# Autodesk Inventor assembly: Winch Assembly
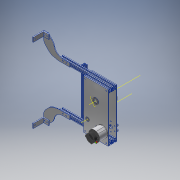
[picture p0: Inventor's stored thumbnail of the model, 180x180]
Saved by Autodesk Inventor 2019.4 (Build 234330000, 330)
## iProperties
Created: 2020-01-24
Part Number: Winch Assembly
Document SubType Name: Assembly
Designer: Mark
Mass: 3605.21 g
Surface Area: 5054.36 cm^2
Volume: 1017.6 cm^3
Density: 3.54284 g/cm^3
Author: Mark
## Documents named in this file (25)
- C:\Users\admin\Desktop\FRC 2020 Engineering\GitHub\7738-2020\Ratchet Winch\Winch Assembly.iam
- C:\Users\admin\Desktop\FRC 2020 Engineering\GitHub\7738-2020\Ratchet Winch\An Extrusion.ipt
- C:\Users\admin\Desktop\FRC 2020 Engineering\GitHub\7738-2020\Elevator MK2\Bottom Pneumatic Extrusion.ipt
- C:\Users\admin\Desktop\FRC 2020 Engineering\GitHub\7738-2020\Ratchet Winch\Support Plate.ipt
- C:\Users\admin\Desktop\FRC 2020 Engineering\GitHub\7738-2020\Ratchet Winch\Small connector.ipt
- C:\Users\admin\Desktop\FRC 2020 Engineering\GitHub\7738-2020\Ratchet Winch\V2 Plate 1.ipt
- C:\Users\admin\Desktop\FRC 2020 Engineering\GitHub\7738-2020\Ratchet Winch\Falcon_500_Powered_by_Talon_FX_217-6515.ipt
- C:\Users\admin\Desktop\FRC 2020 Engineering\GitHub\7738-2020\Robot V2\Turret\F6800.ipt
- C:\Users\admin\Desktop\FRC 2020 Engineering\GitHub\7738-2020\Ratchet Winch\Winch Stopper Stage.ipt
- C:\Users\admin\Desktop\FRC 2020 Engineering\GitHub\7738-2020\CAD\Gearbox\40t_Aluminum_Spur_Gear_20_DP_1_2_Hex_Bore_217-2708.ipt
- C:\Users\admin\Desktop\FRC 2020 Engineering\GitHub\7738-2020\Ratchet Winch\csk15.ipt
- C:\Users\admin\Desktop\FRC 2020 Engineering\GitHub\7738-2020\CAD\Gearbox\10T_Steel_Spur_Gear_20_DP_12T_Center_Distance_Falcon_Motor_217-6917.ipt
- C:\Users\admin\Desktop\FRC 2020 Engineering\GitHub\7738-2020\Ratchet Winch\Winch Assembly\Design Accelerator\Key Connection2.iam
- C:\Users\admin\Desktop\FRC 2020 Engineering\GitHub\7738-2020\Ratchet Winch\Stopper Outer.ipt
- C:\Users\admin\Desktop\FRC 2020 Engineering\GitHub\7738-2020\Ratchet Winch\Stopper Screw Point.ipt
- C:\Users\admin\Desktop\FRC 2020 Engineering\GitHub\7738-2020\Ratchet Winch\Winch Assembly\Design Accelerator\Spur Gears3.iam
- C:\Users\admin\Desktop\FRC 2020 Engineering\GitHub\7738-2020\Ratchet Winch\Winch Assembly\Design Accelerator\Key Connection4.iam
- C:\Users\admin\Desktop\FRC 2020 Engineering\GitHub\7738-2020\Ratchet Winch\F6801.ipt
- C:\Users\admin\Desktop\FRC 2020 Engineering\GitHub\7738-2020\Ratchet Winch\Winch Assembly\Design Accelerator\Shaft1.iam
- C:\Users\admin\Desktop\FRC 2020 Engineering\GitHub\7738-2020\Ratchet Winch\Winch Assembly\Design Accelerator\Synchronous Belts Transmission1.iam
- C:\Users\admin\Desktop\FRC 2020 Engineering\GitHub\7738-2020\CAD\F6804zz.ipt
- C:\Users\admin\Desktop\FRC 2020 Engineering\GitHub\7738-2020\Ratchet Winch\Final Shaft.ipt
- C:\Users\admin\Desktop\FRC 2020 Engineering\GitHub\7738-2020\Ratchet Winch\Winch Assembly\Design Accelerator\Key Connection3.iam
- C:\Users\admin\Desktop\FRC 2020 Engineering\GitHub\7738-2020\Ratchet Winch\Winch Assembly\Design Accelerator\Key Connection5.iam
- C:\Users\admin\Desktop\FRC 2020 Engineering\GitHub\7738-2020\Ratchet Winch\Extrusion Spacer.ipt
## Components (32 placed, 21 different names)
1. An Extrusion:1 — Mate:23, Flush:6, Flush:7, Flush:15, Mate:44, Flush:35, Flush:36, Mate:80
2. An Extrusion:2 — Mate:23, Flush:6, Flush:7, Mate:24, Flush:8, Flush:9, Mate:43, Flush:13, Flush:14, Mate:49, Flush:21, Flush:22, Flush:33, Flush:34, Mate:79
3. Bottom Pneumatic Extrusion:1 — Mate:24, Flush:8, Flush:9
4. Support Plate:1 — Mate:43, Flush:13, Flush:14, Flush:16, Mate:45, Flush:17, Flush:18
5. Support Plate:2 — Flush:15, Mate:44, Flush:16, Flush:19, Flush:20, Mate:46
6. Small connector:1 — Mate:45, Flush:17, Flush:18
7. Small connector:2 — Flush:19, Flush:20, Mate:46
8. V2 Plate 1:1 — Mate:49, Flush:21, Flush:22, Flush:23, Flush:24, Mate:50, Mate:53, Mate:54, Mate:64, Mate:65, Mate:66, Mate:69, Mate:70, Mate:74, Mate:75
9. V2 Plate 1:2 — Flush:23, Flush:24, Mate:50, Mate:51, Mate:52, Mate:55, Mate:56, Flush:25, Mate:71, Mate:72, Flush:30, Mate:76, Mate:77, Flush:31
10. Falcon_500_Powered_by_Talon_FX_217-6515:1 — Mate:51, Mate:52, Mate:62
11. F6800:1 — Mate:53, Mate:54
12. F6800:2 — Mate:55, Mate:56, Mate:57
13. Winch Stopper Stage:1 — Mate:57, Flush:25, Mate:59, Mate:60, Flush:26, Flush:28, Mate:68, Flush:29
14. 40t_Aluminum_Spur_Gear_20_DP_1_2_Hex_Bore_217-2708:1 — Mate:59, Flush:28, Flush:32
15. csk10:1 — Mate:60, Flush:26, Mate:63, Flush:27
16. 10T_Steel_Spur_Gear_20_DP_12T_Center_Distance_Falcon_Motor_217-6917:1 — Mate:62, Flush:32
17. Key Connection:2 [sub-assembly]
18. Stopper Outer:1 — Mate:63, Flush:27, Mate:67
19. Stopper Screw Point:1 — Mate:64, Mate:65, Mate:66
20. Spur Gears:3 [sub-assembly] — Mate:68, Flush:29
21. Key Connection:3 [sub-assembly]
22. F6801:1 — Mate:69, Mate:70
23. F6801:2 — Mate:71, Mate:72, Mate:73
24. Shaft:1 [sub-assembly] — Mate:73, Flush:30
25. Synchronous Belts Transmission:1 [sub-assembly]
26. F6804zz:1 — Mate:74, Mate:75
27. F6804zz:2 — Mate:76, Mate:77, Mate:78
28. Final Shaft:1 — Mate:78, Flush:31
29. Key Connection:4 [sub-assembly]
30. Key Connection:5 [sub-assembly]
31. Extrusion Spacer:1 — Flush:33, Flush:34, Mate:79
32. Extrusion Spacer:2 — Flush:35, Flush:36, Mate:80
## Relationships (64: Mate 36, Flush 28)
- Mate:23 (239 mm): An Extrusion:1 ↔ An Extrusion:2
- Flush:6: An Extrusion:1 ↔ An Extrusion:2
- Flush:7: An Extrusion:1 ↔ An Extrusion:2
- Mate:24: An Extrusion:2 ↔ Bottom Pneumatic Extrusion:1
- Flush:8 (100 mm): An Extrusion:2 ↔ Bottom Pneumatic Extrusion:1
- Flush:9: An Extrusion:2 ↔ Bottom Pneumatic Extrusion:1
- Mate:43: An Extrusion:2 ↔ Support Plate:1
- Flush:13: An Extrusion:2 ↔ Support Plate:1
- Flush:14 (-90 mm): An Extrusion:2 ↔ Support Plate:1
- Flush:15: An Extrusion:1 ↔ Support Plate:2
- Mate:44: An Extrusion:1 ↔ Support Plate:2
- Flush:16: Support Plate:1 ↔ Support Plate:2
- Mate:45: Support Plate:1 ↔ Small connector:1
- Flush:17: Support Plate:1 ↔ Small connector:1
- Flush:18: Support Plate:1 ↔ Small connector:1
- Flush:19: Support Plate:2 ↔ Small connector:2
- Flush:20: Support Plate:2 ↔ Small connector:2
- Mate:46: Support Plate:2 ↔ Small connector:2
- Mate:49: An Extrusion:2 ↔ V2 Plate 1:1
- Flush:21: An Extrusion:2 ↔ V2 Plate 1:1
- Flush:22: An Extrusion:2 ↔ V2 Plate 1:1
- Flush:23: V2 Plate 1:1 ↔ V2 Plate 1:2
- Flush:24: V2 Plate 1:1 ↔ V2 Plate 1:2
- Mate:50 (40 mm): V2 Plate 1:1 ↔ V2 Plate 1:2
- Mate:51: V2 Plate 1:2 ↔ Falcon_500_Powered_by_Talon_FX_217-6515:1
- Mate:52: V2 Plate 1:2 ↔ Falcon_500_Powered_by_Talon_FX_217-6515:1
- Mate:53: V2 Plate 1:1 ↔ F6800:1
- Mate:54: V2 Plate 1:1 ↔ F6800:1
- Mate:55: V2 Plate 1:2 ↔ F6800:2
- Mate:56: V2 Plate 1:2 ↔ F6800:2
- Mate:57: F6800:2 ↔ Winch Stopper Stage:1
- Flush:25: V2 Plate 1:2 ↔ Winch Stopper Stage:1
- Mate:59: Winch Stopper Stage:1 ↔ 40t_Aluminum_Spur_Gear_20_DP_1_2_Hex_Bore_217-2708:1
- Mate:60: Winch Stopper Stage:1 ↔ csk10:1
- Mate:62: Falcon_500_Powered_by_Talon_FX_217-6515:1 ↔ 10T_Steel_Spur_Gear_20_DP_12T_Center_Distance_Falcon_Motor_217-6917:1
- Flush:26 (0.1 mm): Winch Stopper Stage:1 ↔ csk10:1
- Mate:63: csk10:1 ↔ Stopper Outer:1
- Flush:27 (-2.35 mm): csk10:1 ↔ Stopper Outer:1
- Mate:64: V2 Plate 1:1 ↔ Stopper Screw Point:1
- Mate:65: V2 Plate 1:1 ↔ Stopper Screw Point:1
- Mate:66: V2 Plate 1:1 ↔ Stopper Screw Point:1
- Mate:67: Stopper Outer:1
- Flush:28: Winch Stopper Stage:1 ↔ 40t_Aluminum_Spur_Gear_20_DP_1_2_Hex_Bore_217-2708:1
- Mate:68: Winch Stopper Stage:1 ↔ Spur Gears:3
- Flush:29 (0.1 mm): Winch Stopper Stage:1 ↔ Spur Gears:3
- Mate:69: V2 Plate 1:1 ↔ F6801:1
- Mate:70: V2 Plate 1:1 ↔ F6801:1
- Mate:71: V2 Plate 1:2 ↔ F6801:2
- Mate:72: V2 Plate 1:2 ↔ F6801:2
- Mate:73: F6801:2 ↔ Shaft:1
- Flush:30: V2 Plate 1:2 ↔ Shaft:1
- Mate:74: V2 Plate 1:1 ↔ F6804zz:1
- Mate:75: V2 Plate 1:1 ↔ F6804zz:1
- Mate:76: V2 Plate 1:2 ↔ F6804zz:2
- Mate:77: V2 Plate 1:2 ↔ F6804zz:2
- Mate:78: F6804zz:2 ↔ Final Shaft:1
- Flush:31: V2 Plate 1:2 ↔ Final Shaft:1
- Flush:32: 40t_Aluminum_Spur_Gear_20_DP_1_2_Hex_Bore_217-2708:1 ↔ 10T_Steel_Spur_Gear_20_DP_12T_Center_Distance_Falcon_Motor_217-6917:1
- Flush:33: An Extrusion:2 ↔ Extrusion Spacer:1
- Flush:34: An Extrusion:2 ↔ Extrusion Spacer:1
- Mate:79: An Extrusion:2 ↔ Extrusion Spacer:1
- Flush:35: An Extrusion:1 ↔ Extrusion Spacer:2
- Flush:36: An Extrusion:1 ↔ Extrusion Spacer:2
- Mate:80: An Extrusion:1 ↔ Extrusion Spacer:2
